# Autodesk Inventor assembly: suspensionUnit
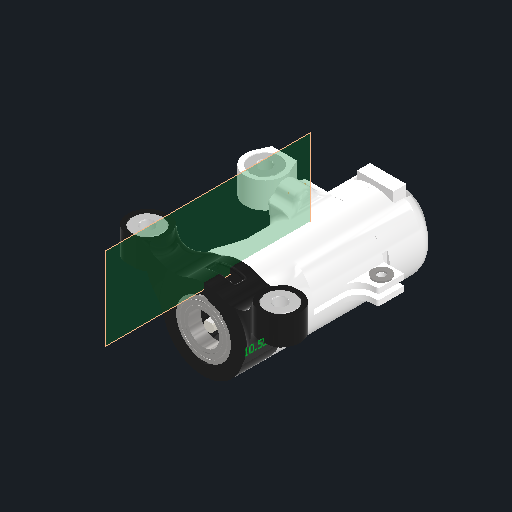
[picture p0: Inventor's stored thumbnail of the model, 512x512]
Saved by Autodesk Inventor 2025 (Build 290162000, 162)
## iProperties
Created: 2023-06-25
Part Number: suspensionUnit
Document SubType Name: Assembly
Designer: khrip
Mass: 147.431 g
Surface Area: 305.3 cm^2
Volume: 59.2335 cm^3
Density: 2.48897 g/cm^3
Author: khrip
## Documents named in this file (13)
- H:\Potamon\OutdatedVersions\suspensionUnit\suspensionUnit.iam
- H:\Potamon\OutdatedVersions\suspensionUnit\servo.ipt
- H:\Potamon\OutdatedVersions\suspensionUnit\bearing.ipt
- C:\Users\khrip\OneDrive\Документы\Inventor\Content Center Files\R2023\ru-RU\DIN 913\DIN 913 - M3 x 4.ipt
- H:\Potamon\OutdatedVersions\suspensionUnit\servoCushion.ipt
- H:\Potamon\OutdatedVersions\suspensionUnit\servoCushionSleeve.ipt
- H:\Potamon\OutdatedVersions\suspensionUnit\sleeve.ipt
- C:\Users\khrip\OneDrive\Документы\Inventor\Content Center Files\R2023\ru-RU\BS EN ISO 7045 H\EN ISO 7045 - M3 x 10 - 4.8 - H(1).ipt
- C:\Users\khrip\Documents\Inventor\Content Center Files\R2025\ru-RU\GOST 11371-78  A\Шайба 3 ГОСТ 11371-78.ipt
- C:\Users\khrip\OneDrive\Документы\Inventor\Content Center Files\R2023\ru-RU\DIN 934\DIN 934 - M3 x 0,5.ipt
- C:\Users\khrip\OneDrive\Документы\Inventor\Content Center Files\R2023\ru-RU\GOST 17475-80 (2)\Винт 2.M3-6gx12 ГОСТ 17475-80.ipt
- H:\Potamon\OutdatedVersions\suspensionUnit\EncCoverHalf.ipt
- H:\Potamon\OutdatedVersions\suspensionUnit\EncCoverHalfMirrored.ipt
## Components (15 placed, 12 different names)
1. servo:1 — Заподлицо:1, Совмещение:6, Совмещение:7, Совмещение:8, Совмещение:9, Совмещение:30, Угол:1, Совмещение:33
2. bearing:1 — Совмещение:10, Совмещение:11
3. DIN 913 M3 x 4:1 — Совмещение:6
4. servoCushion:1 — Совмещение:7, Совмещение:8, Совмещение:9, Заподлицо:2, Совмещение:10, Совмещение:11, Совмещение:12, Совмещение:13, Совмещение:16, Совмещение:17, Совмещение:28, Совмещение:29
5. servoCushionSleeve:1 — Заподлицо:2, Совмещение:14, Совмещение:15, Совмещение:18, Совмещение:19, Совмещение:23, Совмещение:31, Совмещение:34
6. sleeve:1 — Совмещение:14, Совмещение:15
7. sleeve:2 — Совмещение:12, Совмещение:16
8. sleeve:3 — Совмещение:13, Совмещение:17
9. BS EN ISO 7045 H - метрическая M3 x 10 - 4.8 - H:1 — Совмещение:18, Совмещение:19, Совмещение:22, Совмещение:26
10. Шайба  ГОСТ 11371-78 3,2:1 — Совмещение:22, Совмещение:23, Совмещение:27
11. DIN 934 - заменено на DIN EN 24032/28673/28674 M3:1 — Совмещение:26, Совмещение:27
12. Винт 2 ГОСТ 17475-80 M3 x 12:1 — Совмещение:28
13. Винт 2 ГОСТ 17475-80 M3 x 12:2 — Совмещение:29
14. EncCoverHalf:1 — Совмещение:30, Угол:1, Совмещение:31, Совмещение:32
15. EncCoverHalfMirrored:1 — Совмещение:32, Совмещение:33, Совмещение:34
## Relationships (28: Mate 25, Flush 2, Angle 1)
- Заподлицо:1 [Flush]: servo:1
- Совмещение:6 [Mate]: servo:1 ↔ DIN 913 M3 x 4:1
- Совмещение:7 [Mate]: servo:1 ↔ servoCushion:1
- Совмещение:8 [Mate]: servo:1 ↔ servoCushion:1
- Совмещение:9 [Mate]: servo:1 ↔ servoCushion:1
- Заподлицо:2 [Flush]: servoCushion:1 ↔ servoCushionSleeve:1
- Совмещение:10 [Mate]: bearing:1 ↔ servoCushion:1
- Совмещение:11 [Mate]: bearing:1 ↔ servoCushion:1
- Совмещение:12 [Mate]: servoCushion:1 ↔ sleeve:2
- Совмещение:13 [Mate]: servoCushion:1 ↔ sleeve:3
- Совмещение:14 [Mate]: servoCushionSleeve:1 ↔ sleeve:1
- Совмещение:15 [Mate]: servoCushionSleeve:1 ↔ sleeve:1
- Совмещение:16 [Mate]: servoCushion:1 ↔ sleeve:2
- Совмещение:17 [Mate]: servoCushion:1 ↔ sleeve:3
- Совмещение:18 [Mate]: servoCushionSleeve:1 ↔ BS EN ISO 7045 H - метрическая M3 x 10 - 4.8 - H:1
- Совмещение:19 [Mate]: servoCushionSleeve:1 ↔ BS EN ISO 7045 H - метрическая M3 x 10 - 4.8 - H:1
- Совмещение:22 [Mate]: BS EN ISO 7045 H - метрическая M3 x 10 - 4.8 - H:1 ↔ Шайба  ГОСТ 11371-78 3,2:1
- Совмещение:23 [Mate]: servoCushionSleeve:1 ↔ Шайба  ГОСТ 11371-78 3,2:1
- Совмещение:26 [Mate]: BS EN ISO 7045 H - метрическая M3 x 10 - 4.8 - H:1 ↔ DIN 934 - заменено на DIN EN 24032/28673/28674 M3:1
- Совмещение:27 [Mate]: Шайба  ГОСТ 11371-78 3,2:1 ↔ DIN 934 - заменено на DIN EN 24032/28673/28674 M3:1
- Совмещение:28 [Mate]: servoCushion:1 ↔ Винт 2 ГОСТ 17475-80 M3 x 12:1
- Совмещение:29 [Mate]: servoCushion:1 ↔ Винт 2 ГОСТ 17475-80 M3 x 12:2
- Совмещение:30 [Mate]: servo:1 ↔ EncCoverHalf:1
- Угол:1 [Angle] (180 deg): servo:1 ↔ EncCoverHalf:1
- Совмещение:31 [Mate]: servoCushionSleeve:1 ↔ EncCoverHalf:1
- Совмещение:32 [Mate]: EncCoverHalf:1 ↔ EncCoverHalfMirrored:1
- Совмещение:33 [Mate]: servo:1 ↔ EncCoverHalfMirrored:1
- Совмещение:34 [Mate]: servoCushionSleeve:1 ↔ EncCoverHalfMirrored:1
